# Autodesk Inventor assembly: Butler_assembly
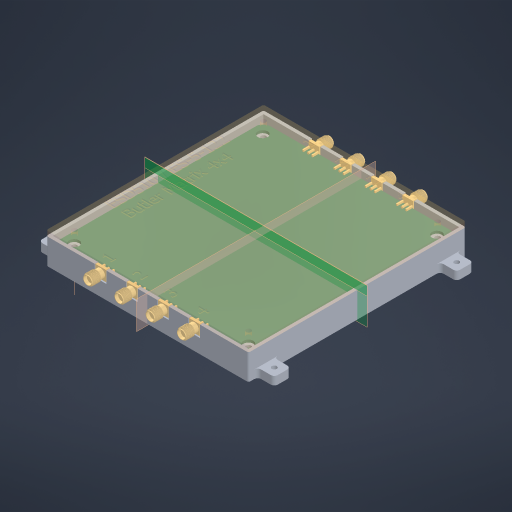
[picture p0: Inventor's stored thumbnail of the model, 512x512]
Saved by Autodesk Inventor 2023.4 (Build 274418000, 418)
## iProperties
Created: 2025-10-09
Part Number: Butler_assembly
Document SubType Name: Assembly
Designer: Mikke
Author: Mikke
## Documents named in this file (4)
- C:\Users\Malthe Sennels\OneDrive - Aalborg Universitet\ESD 510 - General\Projekt\Inventor\Butler_matrix\Butler_assembly.iam
- C:\Users\Malthe Sennels\OneDrive - Aalborg Universitet\ESD 510 - General\Projekt\Inventor\Butler_matrix\Case.ipt
- C:\Users\Malthe Sennels\OneDrive - Aalborg Universitet\ESD 510 - General\Projekt\Inventor\Butler_matrix\Butler_matrix\Butler_matrix.ipt
- C:\Users\Malthe Sennels\OneDrive - Aalborg Universitet\ESD 510 - General\Projekt\Inventor\Butler_matrix\Cover_acryl.ipt
## Components (3 placed, 3 different names)
1. Case:1 — Mate:1, Mate:2, Mate:3, Flush:1, Flush:2, Mate:4
2. Butler_matrix:1 — Mate:1, Mate:2, Mate:3
3. Cover_acryl:1 — Flush:1, Flush:2, Mate:4
## Relationships (6: Mate 4, Flush 2)
- Mate:1: Case:1 ↔ Butler_matrix:1
- Mate:2: Case:1 ↔ Butler_matrix:1
- Mate:3: Case:1 ↔ Butler_matrix:1
- Flush:1: Case:1 ↔ Cover_acryl:1
- Flush:2: Case:1 ↔ Cover_acryl:1
- Mate:4: Case:1 ↔ Cover_acryl:1
